# Autodesk Inventor assembly: ASY PNS FDS way1_1600
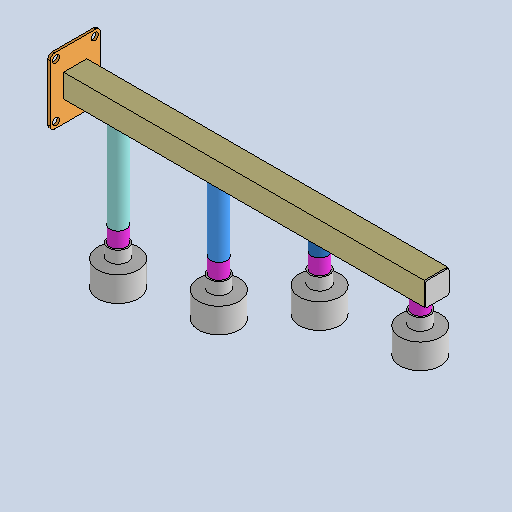
[picture p0: Inventor's stored thumbnail of the model, 512x512]
Saved by Autodesk Inventor 2025 (Build 290162010, 162A)
## iProperties
Created: 2025-07-02
Part Number: ASY PNS FDS way1_1600
Document SubType Name: Assembly
Designer: admin
Author: user
## Documents named in this file (9)
- C:\Users\admin\Yandex.Disk\home pc\Inventor\PNS2-Panaevsk\Filter D1000\filter-distribution-system 1000\ASY PNS FDS way1_1600.iam
- C:\Users\admin\Yandex.Disk\home pc\Inventor\PNS2-Panaevsk\Filter D1000\filter-distribution-system 1000\PNS 754 FDS 1200 way tube 1_1600.ipt
- C:\Users\admin\Yandex.Disk\home pc\Inventor\PNS2-Panaevsk\Filter D1000\filter-distribution-system 1000\PNS dummy filter element_1600.ipt
- C:\Users\admin\Yandex.Disk\home pc\Inventor\PNS2-Panaevsk\Filter D1000\filter-distribution-system 1000\PNS dummy pipe nippel_1600.ipt
- C:\Users\admin\Yandex.Disk\home pc\Inventor\PNS2-Panaevsk\Filter D1000\filter-distribution-system 1000\PNS 757 FDS 1200 way tube 4_1600.ipt
- C:\Users\admin\Yandex.Disk\home pc\Inventor\PNS2-Panaevsk\Filter D1000\filter-distribution-system 1000\PNS 1756 FDS 1200 way tube 6_1600.ipt
- C:\Users\admin\Yandex.Disk\home pc\Inventor\PNS2-Panaevsk\Filter D1000\filter-distribution-system 1000\PNS 1757 FDS 1200 way tube 7_1600.ipt
- C:\Users\admin\Yandex.Disk\home pc\Inventor\PNS2-Panaevsk\Filter D1000\filter-distribution-system 1000\PNS 760 FDS 1200 FLANGE 3_1600.ipt
- C:\Users\admin\Yandex.Disk\home pc\Inventor\PNS2-Panaevsk\Filter D1000\filter-distribution-system 1000\PNS 766 FDS 1200 CUP 1_1600.ipt
## Components (14 placed, 8 different names)
1. PNS 754 FDS 1200 way tube 1_1600:1 — Rigid:2, Rigid:5, Rigid:10, Rigid:11, Rigid:12, Rigid:13
2. PNS dummy filter element_1600:1 — Rigid:1
3. PNS dummy pipe nippel_1600:1 — Rigid:2, Rigid:1
4. PNS 757 FDS 1200 way tube 4_1600:1 — Rigid:5, Rigid:4
5. PNS dummy filter element_1600:2 — Rigid:3
6. PNS dummy pipe nippel_1600:2 — Rigid:4, Rigid:3
7. PNS 1756 FDS 1200 way tube 6_1600:1 — Rigid:10, Rigid:7
8. PNS dummy filter element_1600:3 — Rigid:6
9. PNS dummy pipe nippel_1600:3 — Rigid:7, Rigid:6
10. PNS 1757 FDS 1200 way tube 7_1600:1 — Rigid:11, Rigid:9
11. PNS dummy filter element_1600:4 — Rigid:8
12. PNS dummy pipe nippel_1600:4 — Rigid:9, Rigid:8
13. PNS 760 FDS 1200 FLANGE 3_1600:1 — Rigid:12
14. PNS 766 FDS 1200 CUP 1_1600:1 — Rigid:13
## Relationships (13: WeldJoint 13)
- Rigid:2 [WeldJoint]: PNS 754 FDS 1200 way tube 1_1600:1 ↔ PNS dummy pipe nippel_1600:1
- Rigid:1 [WeldJoint]: PNS dummy filter element_1600:1 ↔ PNS dummy pipe nippel_1600:1
- Rigid:5 [WeldJoint]: PNS 754 FDS 1200 way tube 1_1600:1 ↔ PNS 757 FDS 1200 way tube 4_1600:1
- Rigid:4 [WeldJoint]: PNS 757 FDS 1200 way tube 4_1600:1 ↔ PNS dummy pipe nippel_1600:2
- Rigid:3 [WeldJoint]: PNS dummy filter element_1600:2 ↔ PNS dummy pipe nippel_1600:2
- Rigid:10 [WeldJoint]: PNS 754 FDS 1200 way tube 1_1600:1 ↔ PNS 1756 FDS 1200 way tube 6_1600:1
- Rigid:7 [WeldJoint]: PNS 1756 FDS 1200 way tube 6_1600:1 ↔ PNS dummy pipe nippel_1600:3
- Rigid:6 [WeldJoint]: PNS dummy filter element_1600:3 ↔ PNS dummy pipe nippel_1600:3
- Rigid:11 [WeldJoint]: PNS 754 FDS 1200 way tube 1_1600:1 ↔ PNS 1757 FDS 1200 way tube 7_1600:1
- Rigid:9 [WeldJoint]: PNS 1757 FDS 1200 way tube 7_1600:1 ↔ PNS dummy pipe nippel_1600:4
- Rigid:8 [WeldJoint]: PNS dummy filter element_1600:4 ↔ PNS dummy pipe nippel_1600:4
- Rigid:12 [WeldJoint] (-2 mm): PNS 754 FDS 1200 way tube 1_1600:1 ↔ PNS 760 FDS 1200 FLANGE 3_1600:1
- Rigid:13 [WeldJoint]: PNS 754 FDS 1200 way tube 1_1600:1 ↔ PNS 766 FDS 1200 CUP 1_1600:1
